# Autodesk Inventor assembly: Illumination Assembly with Posts
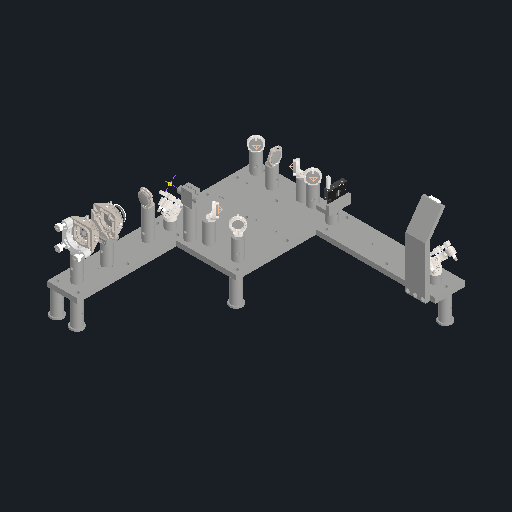
[picture p0: Inventor's stored thumbnail of the model, 512x512]
Saved by Autodesk Inventor 2026 (Build 300175000, 175)
## iProperties
Created: 2026-03-03
Part Number: Illumination Assembly with Posts
Document SubType Name: Assembly
Designer: FiolkaLab
Author: FiolkaLab
## Documents named in this file (4)
- E:\Muaaz\Baseplate\Illumination\Illumination Assembly with Posts.iam
- E:\Muaaz\Baseplate\Illumination\Baseplate Illum V3 L Assembly.iam
- E:\Muaaz\Baseplate\Illumination\RS2.5P-Step\RS2.5P-Step\RS2.5P-Step.ipt
- E:\Muaaz\Baseplate\ASLM_DvOPM System Assembly\RS2.5P-Step\RS2.5P-Step\RS2.5P-Step.ipt
## Components (20 placed, 2 different names)
1. Baseplate Illum V3 L Assembly:1 [sub-assembly] — Mate:3, Mate:4, Mate:5, Mate:6, Mate:7, Mate:8, Mate:10, Mate:11, Mate:14, Mate:15, Mate:17, Mate:18, Mate:19, Mate:20, Mate:24, Mate:25, Mate:26, Mate:28, Mate:29, Mate:30, Mate:31, Mate:32, Mate:35, Mate:36, Mate:37, Mate:38, Mate:39, Mate:40, Mate:41, Mate:42, Mate:43, Mate:44, Mate:45, Mate:46, Mate:47, Mate:48, Mate:49, Mate:50
2. RS2.5P-Step:1 — Mate:3, Mate:4
3. RS2.5P-Step:2 — Mate:6, Mate:29
4. RS2.5P-Step:4 — Mate:11, Mate:38
5. RS2.5P-Step:6 — Mate:15, Mate:26
6. RS2.5P-Step:8 — Mate:17, Mate:32
7. RS2.5P-Step:9 — Mate:18, Mate:31
8. RS2.5P-Step:10 — Mate:20, Mate:25
9. RS2.5P-Step:12 — Mate:19, Mate:30
10. RS2.5P-Step:13 — Mate:14, Mate:24
11. RS2.5P-Step:15 — Mate:10, Mate:35
12. RS2.5P-Step:16 — Mate:7, Mate:36
13. RS2.5P-Step:18 — Mate:5, Mate:37
14. RS2.5P-Step:19 — Mate:8, Mate:28
15. RS2.5P-Step:20 — Mate:44, Mate:50
16. RS2.5P-Step:21 — Mate:40, Mate:46
17. RS2.5P-Step:22 — Mate:42, Mate:47
18. RS2.5P-Step:23 — Mate:41, Mate:48
19. RS2.5P-Step:24 — Mate:43, Mate:49
20. RS2.5P-Step:25 — Mate:39, Mate:45
## Relationships (38: Mate 38)
- Mate:3: Baseplate Illum V3 L Assembly:1 ↔ RS2.5P-Step:1
- Mate:4: Baseplate Illum V3 L Assembly:1 ↔ RS2.5P-Step:1
- Mate:5: Baseplate Illum V3 L Assembly:1 ↔ RS2.5P-Step:18
- Mate:6: Baseplate Illum V3 L Assembly:1 ↔ RS2.5P-Step:2
- Mate:7: Baseplate Illum V3 L Assembly:1 ↔ RS2.5P-Step:16
- Mate:8: Baseplate Illum V3 L Assembly:1 ↔ RS2.5P-Step:19
- Mate:10: Baseplate Illum V3 L Assembly:1 ↔ RS2.5P-Step:15
- Mate:11: Baseplate Illum V3 L Assembly:1 ↔ RS2.5P-Step:4
- Mate:14: Baseplate Illum V3 L Assembly:1 ↔ RS2.5P-Step:13
- Mate:15: Baseplate Illum V3 L Assembly:1 ↔ RS2.5P-Step:6
- Mate:17: Baseplate Illum V3 L Assembly:1 ↔ RS2.5P-Step:8
- Mate:18: Baseplate Illum V3 L Assembly:1 ↔ RS2.5P-Step:9
- Mate:19: Baseplate Illum V3 L Assembly:1 ↔ RS2.5P-Step:12
- Mate:20: Baseplate Illum V3 L Assembly:1 ↔ RS2.5P-Step:10
- Mate:24: Baseplate Illum V3 L Assembly:1 ↔ RS2.5P-Step:13
- Mate:25: Baseplate Illum V3 L Assembly:1 ↔ RS2.5P-Step:10
- Mate:26: Baseplate Illum V3 L Assembly:1 ↔ RS2.5P-Step:6
- Mate:28: Baseplate Illum V3 L Assembly:1 ↔ RS2.5P-Step:19
- Mate:29: Baseplate Illum V3 L Assembly:1 ↔ RS2.5P-Step:2
- Mate:30: Baseplate Illum V3 L Assembly:1 ↔ RS2.5P-Step:12
- Mate:31: Baseplate Illum V3 L Assembly:1 ↔ RS2.5P-Step:9
- Mate:32: Baseplate Illum V3 L Assembly:1 ↔ RS2.5P-Step:8
- Mate:35: Baseplate Illum V3 L Assembly:1 ↔ RS2.5P-Step:15
- Mate:36: Baseplate Illum V3 L Assembly:1 ↔ RS2.5P-Step:16
- Mate:37: Baseplate Illum V3 L Assembly:1 ↔ RS2.5P-Step:18
- Mate:38: Baseplate Illum V3 L Assembly:1 ↔ RS2.5P-Step:4
- Mate:39: Baseplate Illum V3 L Assembly:1 ↔ RS2.5P-Step:25
- Mate:40: Baseplate Illum V3 L Assembly:1 ↔ RS2.5P-Step:21
- Mate:41: Baseplate Illum V3 L Assembly:1 ↔ RS2.5P-Step:23
- Mate:42: Baseplate Illum V3 L Assembly:1 ↔ RS2.5P-Step:22
- Mate:43: Baseplate Illum V3 L Assembly:1 ↔ RS2.5P-Step:24
- Mate:44: Baseplate Illum V3 L Assembly:1 ↔ RS2.5P-Step:20
- Mate:45: Baseplate Illum V3 L Assembly:1 ↔ RS2.5P-Step:25
- Mate:46: Baseplate Illum V3 L Assembly:1 ↔ RS2.5P-Step:21
- Mate:47: Baseplate Illum V3 L Assembly:1 ↔ RS2.5P-Step:22
- Mate:48: Baseplate Illum V3 L Assembly:1 ↔ RS2.5P-Step:23
- Mate:49: Baseplate Illum V3 L Assembly:1 ↔ RS2.5P-Step:24
- Mate:50: Baseplate Illum V3 L Assembly:1 ↔ RS2.5P-Step:20
